# Autodesk Inventor assembly: Static Parts Assembly
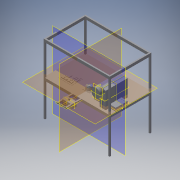
[picture p0: Inventor's stored thumbnail of the model, 180x180]
Saved by Autodesk Inventor 2019 (Build 230136000, 136)
## iProperties
Created: 2021-05-09
Part Number: Static Parts Assembly
Document SubType Name: Assembly
Designer: Eric
Author: Eric
## Documents named in this file (6)
- C:\Users\Eric\Documents\! - Uni\Year 4\MENG-Robot-Fab-Project\Models\For_Optimiser\Static Parts Assembly\Static Parts Assembly.iam
- C:\Users\Eric\Documents\! - Uni\Year 4\MENG-Robot-Fab-Project\Models\For_Optimiser\Static Parts Assembly\RobotFabFrame_3 assembly\RobotFab Frame 3.iam
- C:\Users\Eric\Documents\! - Uni\Year 4\MENG-Robot-Fab-Project\Models\For_Optimiser\Static Parts Assembly\Organ Bank Assembly\Organ Bank Pretty-Convex Assembly.iam
- C:\Users\Eric\Documents\! - Uni\Year 4\MENG-Robot-Fab-Project\Models\For_Optimiser\Static Parts Assembly\TAZ 6 Assembly\TAZ 6 Assembly.iam
- C:\Users\Eric\Documents\! - Uni\Year 4\MENG-Robot-Fab-Project\Models\For_Optimiser\Static Parts Assembly\Assembly Mount Assembly\Assembly Mount Assembly.iam
- C:\Users\Eric\Documents\! - Uni\Year 4\MENG-Robot-Fab-Project\Models\For_Optimiser\Static Parts Assembly\Arm base assembly\ArmBaseAssembly.iam
## Components (5 placed, 5 different names)
1. RobotFab Frame 3:1 [sub-assembly] — Mate:1, Flush:1, Flush:2, Flush:3, Flush:4, Mate:2, Mate:12, Flush:6, Mate:11, Mate:5, Flush:9, Mate:8, Angle:1, Mate:10
2. Organ Bank Pretty-Convex Assembly:1 [sub-assembly] — Flush:3, Flush:4, Mate:2
3. TAZ 6 Assembly:1 [sub-assembly] — Mate:12, Flush:6, Mate:11
4. Assembly Mount Assembly:1 [sub-assembly] — Mate:5, Flush:9, Mate:8
5. ArmBaseAssembly:1 [sub-assembly] — Mate:9, Angle:1, Mate:10
## Relationships (15: Mate 8, Flush 6, Angle 1)
- Mate:1 (260 mm): RobotFab Frame 3:1
- Flush:1 (-10 mm): RobotFab Frame 3:1
- Flush:2 (125.35 mm): RobotFab Frame 3:1
- Flush:3 (51 mm): RobotFab Frame 3:1 ↔ Organ Bank Pretty-Convex Assembly:1
- Flush:4 (550 mm): RobotFab Frame 3:1 ↔ Organ Bank Pretty-Convex Assembly:1
- Mate:2 (260 mm): RobotFab Frame 3:1 ↔ Organ Bank Pretty-Convex Assembly:1
- Mate:12 (263.783 mm): RobotFab Frame 3:1 ↔ TAZ 6 Assembly:1
- Flush:6 (-90.715 mm): RobotFab Frame 3:1 ↔ TAZ 6 Assembly:1
- Mate:11 (662.5 mm): RobotFab Frame 3:1 ↔ TAZ 6 Assembly:1
- Mate:5: RobotFab Frame 3:1 ↔ Assembly Mount Assembly:1
- Flush:9: RobotFab Frame 3:1 ↔ Assembly Mount Assembly:1
- Mate:8: RobotFab Frame 3:1 ↔ Assembly Mount Assembly:1
- Mate:9: ArmBaseAssembly:1
- Angle:1 (0 deg): RobotFab Frame 3:1 ↔ ArmBaseAssembly:1
- Mate:10: RobotFab Frame 3:1 ↔ ArmBaseAssembly:1
